# Autodesk Inventor assembly: printer
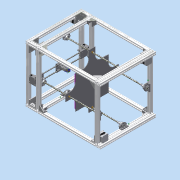
[picture p0: Inventor's stored thumbnail of the model, 180x180]
Saved by Autodesk Inventor 2015 (Build 190159000, 159)
## iProperties
Created: 2016-06-24
Part Number: printer
Document SubType Name: Assembly
Designer: Dustin
Author: Dustin
## Documents named in this file (25)
- E:\Documents\3D Printer\LetzteBot3DPrinter\Inventor Files\IAM Files\printer.iam
- E:\Documents\3D Printer\LetzteBot3DPrinter\Inventor Files\IPT Files\AF350.ipt
- E:\Documents\3D Printer\LetzteBot3DPrinter\Inventor Files\IPT Files\AF380.ipt
- E:\Documents\3D Printer\LetzteBot3DPrinter\Inventor Files\IPT Files\HB1.ipt
- E:\Documents\3D Printer\LetzteBot3DPrinter\Inventor Files\IPT Files\NEMA17.ipt
- E:\Documents\3D Printer\LetzteBot3DPrinter\Inventor Files\IPT Files\LS2.ipt
- E:\Documents\3D Printer\LetzteBot3DPrinter\Inventor Files\IPT Files\LSM1.ipt
- E:\Documents\3D Printer\LetzteBot3DPrinter\Inventor Files\IPT Files\BP1.ipt
- E:\Documents\3D Printer\LetzteBot3DPrinter\Inventor Files\IPT Files\Imported Components\GT2_20teeth_pulley\GT2P.ipt
- E:\Documents\3D Printer\LetzteBot3DPrinter\Inventor Files\IPT Files\SR385.ipt
- E:\Documents\3D Printer\LetzteBot3DPrinter\Inventor Files\IPT Files\MM1.ipt
- E:\Documents\3D Printer\LetzteBot3DPrinter\Inventor Files\IPT Files\AF50.ipt
- E:\Documents\3D Printer\LetzteBot3DPrinter\Inventor Files\IAM Files\extruder.iam
- E:\Documents\3D Printer\LetzteBot3DPrinter\Inventor Files\IPT Files\SM1.ipt
- E:\Documents\3D Printer\LetzteBot3DPrinter\Inventor Files\IPT Files\S320.ipt
- E:\Documents\3D Printer\LetzteBot3DPrinter\Inventor Files\IPT Files\CM1.ipt
- E:\Documents\3D Printer\LetzteBot3DPrinter\Inventor Files\IAM Files\M4BA1.iam
- E:\Documents\3D Printer\LetzteBot3DPrinter\Inventor Files\IAM Files\M4BA2.iam
- E:\Documents\3D Printer\LetzteBot3DPrinter\Inventor Files\IAM Files\KFL08.iam
- E:\Documents\3D Printer\LetzteBot3DPrinter\Inventor Files\IAM Files\VW1.iam
- E:\Documents\3D Printer\LetzteBot3DPrinter\Inventor Files\IPT Files\S516.ipt
- E:\Documents\3D Printer\LetzteBot3DPrinter\Inventor Files\IPT Files\LSN1.ipt
- E:\Documents\3D Printer\LetzteBot3DPrinter\Inventor Files\IPT Files\CB2.ipt
- E:\Documents\3D Printer\LetzteBot3DPrinter\Inventor Files\IPT Files\CM2.ipt
- E:\Documents\3D Printer\LetzteBot3DPrinter\Inventor Files\IPT Files\CB1.ipt
## Components (123 placed, 24 different names)
1. NEMA17:1 — Mate:39, Flush:64, Insert:7, Mate:85, Insert:59
2. NEMA17:2 — Flush:65, Insert:6, Insert:20, Insert:21
3. NEMA17:3 — Mate:87, Mate:88, Insert:32, Insert:60
4. NEMA17:4 — Insert:23, Insert:24, Mate:90, Tangent:34, Insert:31, Mate:98
5. CM1:2 — Flush:91, Mate:101, Angle:14, Tangent:38, Flush:94, Angle:15, Tangent:39, Mate:103
6. MM1:2 — Insert:20, Insert:21, Flush:123
7. MM1:3 — Insert:23, Insert:24, Mate:89
8. MM1:4 — Insert:59, Angle:30
9. MM1:5 — Insert:60, Angle:31, Mate:115
10. CB2:5 — Mate:116, Mate:117, Flush:124
11. CB2:6 — Mate:118, Flush:125, Mate:119
12. CB2:7 — Mate:126, Flush:129, Mate:127
13. CB2:8 — Mate:124, Mate:125, Flush:128
14. CB2:9 — Mate:122, Mate:123, Flush:127
15. CB2:10 — Mate:120, Mate:121, Flush:126
16. CB2:11 — Mate:128, Mate:129, Flush:130
17. CB2:12 — Mate:130, Mate:131, Flush:131
18. CM2:1 — Mate:132, Mate:133, Mate:134
19. CB1:1 — Mate:135, Flush:132, Mate:136
20. CB1:2 — Mate:137, Mate:138, Flush:133
21. CB1:3 — Mate:139, Flush:134, Mate:140
22. CB1:4 — Mate:141, Mate:142, Flush:135
23. CB1:5 — Mate:143, Flush:136, Mate:144
24. CB1:6 — Mate:145, Mate:146, Flush:137
25. CB1:7 — Mate:147, Mate:148, Flush:138
26. CB1:8 — Mate:149, Mate:150, Flush:139
27. CB2:1 — Mate:107, Flush:119, Mate:108
28. CB2:2 — Mate:109, Mate:110, Flush:120
29. CB2:3 — Mate:113, Mate:114, Flush:122
30. CB2:4 — Mate:111, Mate:112, Flush:121
31. AF380:11 — Mate:60, Flush:60, Flush:61
32. AF380:12 — Flush:62, Mate:61, Flush:63
33. AF50:1 — Flush:71, Flush:72, Mate:72, Mate:143, Mate:147
34. AF50:2 — Mate:75, Flush:73, Flush:74, Mate:132, Mate:133, Mate:140, Mate:141, Flush:135, Mate:151, Flush:140
35. AF50:3 — Mate:74, Flush:75, Flush:76, Mate:138, Mate:150, Flush:139
36. AF50:4 — Mate:73, Flush:77, Flush:78, Mate:77, Flush:81, Flush:82, Mate:136, Mate:145
37. AF380:13 — Mate:77, Flush:81, Flush:82, Mate:88, Mate:90, Flush:142
38. AF350:7 — Mate:89, Mate:98, Flush:91, Mate:101, Flush:106, Flush:141, Flush:142
39. AF350:8 — Mate:87, Angle:28, Angle:31, Mate:115, Mate:134
40. AF350:2 — Mate:4, Flush:8, Flush:9, Mate:6, Mate:39, Flush:53, Flush:64, Mate:66, Mate:113, Flush:122, Angle:30
41. AF350:3 — Mate:5, Flush:10, Flush:11, Flush:12, Flush:13, Mate:48, Flush:51, Flush:65, Mate:67, Mate:109, Flush:120
42. AF380:3 — Mate:4, Flush:8, Flush:9, Mate:5, Flush:10, Flush:11, Mate:11, Mate:12, Flush:24, Flush:25, Flush:26, Flush:27, Mate:60, Flush:60, Flush:61, Mate:85, Flush:113, Mate:104, Mate:108
43. AF380:4 — Mate:6, Flush:12, Flush:13, Mate:10, Mate:13, Flush:21, Flush:22, Flush:23, Flush:28, Flush:29, Mate:54, Flush:54, Flush:62, Mate:61, Flush:63, Mate:68, Mate:111, Flush:121, Flush:123
44. AF380:5 — Mate:13, Flush:21, Flush:28, Flush:29, Mate:116, Mate:127
45. AF380:6 — Mate:12, Flush:26, Flush:27, Mate:14, Flush:30, Flush:31, Mate:107, Flush:119, Mate:110, Mate:119, Mate:120
46. AF380:7 — Mate:11, Flush:24, Flush:25, Mate:122, Flush:127, Mate:125
47. AF380:8 — Mate:10, Flush:22, Flush:23, Mate:112, Mate:114, Mate:129, Mate:130, Flush:131
48. AF350:5 — Mate:40, Flush:47, Flush:48, Flush:73, Flush:105, Mate:117, Flush:124, Mate:118, Flush:125, Mate:142, Flush:136, Mate:144
49. AF350:6 — Mate:44, Flush:50, Flush:77, Mate:83, Flush:104, Mate:124, Flush:128, Mate:128, Flush:130, Mate:135, Flush:132, Mate:137, Flush:133
50. AF380:9 — Mate:14, Flush:30, Flush:31, Mate:42, Flush:49, Mate:74, Mate:75, Flush:74, Flush:75, Flush:76, Angle:29, Mate:121, Flush:126, Mate:123, Mate:139, Flush:134, Mate:149
51. AF380:10 — Mate:46, Flush:71, Flush:72, Mate:72, Mate:73, Flush:78, Mate:126, Flush:129, Mate:131, Mate:146, Flush:137, Mate:148, Flush:138
52. AF380:14 — Mate:151, Flush:140, Flush:141
53. LSN1:1 — Insert:50, Tangent:73
54. LSN1:2 — Insert:51, Tangent:74
55. LSN1:3 — Insert:52, Tangent:72, Tangent:75
56. LSN1:4 — Mate:106, Insert:58
57. GT2P:1 — Insert:33
58. GT2P:2 — Insert:5
59. GT2P:3 — Insert:3
60. GT2P:4 — Insert:4
61. GT2P:5 — Insert:6
62. GT2P:6 — Insert:7
63. S320:5 — Insert:54
64. S320:6 — Insert:57
65. S320:7 — Insert:56
66. S320:8 — Insert:55
67. KFL08:1 [sub-assembly] — Flush:109, Tangent:53, Tangent:61
68. KFL08:2 [sub-assembly] — Flush:110, Tangent:55, Tangent:63
69. KFL08:3 [sub-assembly] — Flush:111, Tangent:56, Tangent:57
70. KFL08:4 [sub-assembly] — Flush:112, Tangent:58, Tangent:59
71. KFL08:5 [sub-assembly] — Flush:117, Tangent:68, Tangent:69
72. KFL08:6 [sub-assembly] — Flush:118, Tangent:70, Tangent:71
73. KFL08:7 [sub-assembly] — Flush:116, Tangent:66, Tangent:67
74. KFL08:8 [sub-assembly] — Flush:115, Tangent:64, Tangent:65
75. HB1:1 — Mate:58, Tangent:5, Tangent:6, Insert:54, Insert:55, Insert:56, Insert:57
76. LS2:1 — Tangent:1, Flush:58, Insert:3, Tangent:18, Tangent:24, Tangent:56, Tangent:64
77. LS2:2 — Insert:33, Flush:114, Tangent:62, Tangent:63, Tangent:66, Tangent:75
78. LS2:3 — Tangent:3, Flush:56, Insert:5, Tangent:14, Tangent:58, Tangent:60, Tangent:68
79. LS2:4 — Tangent:2, Flush:55, Insert:4, Tangent:16, Tangent:21, Tangent:53, Tangent:70
80. LSM1:1 — Mate:40, Flush:47, Tangent:1, Flush:111, Tangent:57
81. LSM1:2 — Mate:42, Flush:48, Flush:110, Tangent:55
82. LSM1:3 — Mate:44, Flush:49, Tangent:3, Flush:112, Tangent:59
83. LSM1:4 — Mate:46, Flush:50, Tangent:2, Flush:109, Tangent:61
84. LSM1:5 — Mate:48, Flush:51, Flush:58, Tangent:18, Mate:67, Flush:115, Tangent:65
85. LSM1:6 — Flush:113, Mate:104, Flush:114, Tangent:62, Flush:116, Tangent:67
86. LSM1:7 — Mate:54, Flush:54, Flush:55, Tangent:16, Mate:68, Flush:118, Tangent:71
87. LSM1:8 — Flush:53, Flush:56, Tangent:14, Mate:66, Flush:117, Tangent:69
88. BP1:1 — Mate:58, Tangent:5, Tangent:6, Tangent:21, Tangent:24, Tangent:60, Insert:50, Insert:51, Insert:52, Angle:28, Angle:29, Tangent:72, Tangent:73, Tangent:74, Mate:106, Insert:58
89. S320:1 — Tangent:35, Angle:11, Flush:107
90. S320:2 — Tangent:36, Angle:12, Flush:108
91. S320:3 — Angle:21, Tangent:45, Flush:100
92. S320:4 — Angle:22, Tangent:46, Flush:101
93. S516:1 — Insert:40
94. S516:2 — Insert:41
95. S516:3 — Insert:39
96. S516:4 — Insert:38
97. S516:5 — Insert:46
98. S516:6 — Insert:47
99. S516:7 — Insert:49
100. S516:8 — Insert:48
101. VW1:1 [sub-assembly] — Insert:37
102. VW1:4 [sub-assembly] — Insert:35
103. VW1:3 [sub-assembly] — Insert:36
104. VW1:2 [sub-assembly] — Insert:34
105. VW1:5 [sub-assembly] — Insert:42
106. VW1:6 [sub-assembly] — Insert:43
107. VW1:7 [sub-assembly] — Insert:44
108. VW1:8 [sub-assembly] — Insert:45
109. SR385:1 — Flush:68, Mate:83, Tangent:22, Tangent:47, Tangent:51, Angle:26, Angle:27
110. SR385:2 — Flush:68, Tangent:23, Tangent:48, Angle:25, Tangent:52
111. SM1:1 — Angle:13, Tangent:37, Flush:93, Angle:16, Tangent:40, Flush:95, Tangent:51, Angle:25, Flush:104, Tangent:52, Insert:42, Insert:43, Insert:44, Insert:45, Insert:46, Insert:47, Insert:48, Insert:49
112. SM1:2 — Tangent:47, Tangent:48, Tangent:49, Tangent:50, Angle:23, Angle:24, Flush:102, Flush:103, Angle:26, Flush:105, Insert:34, Insert:35, Insert:36, Insert:37, Insert:38, Insert:39, Insert:40, Insert:41
113. extruder:1 [sub-assembly] — Tangent:22, Tangent:23, Tangent:35, Angle:11, Tangent:36, Angle:12, Angle:21, Tangent:45, Angle:22, Tangent:46, Flush:100, Flush:101, Flush:106, Flush:107, Angle:27, Flush:108
114. M4BA1:1 [sub-assembly] — Angle:13, Tangent:37, Flush:93
115. M4BA1:2 [sub-assembly] — Angle:14, Tangent:38, Flush:94
116. M4BA2:1 [sub-assembly] — Angle:15, Tangent:39, Mate:103
117. M4BA2:2 [sub-assembly] — Angle:16, Tangent:40, Flush:95
118. M4BA1:3 [sub-assembly] — Tangent:50, Angle:24, Flush:103
119. M4BA2:3 [sub-assembly] — Tangent:49, Angle:23, Flush:102
120. M4BA1:4 [sub-assembly]
121. M4BA2:4 [sub-assembly]
122. GT2P:7 — Insert:32
123. GT2P:8 — Tangent:34, Insert:31
## Relationships (287: Flush 98, Mate 85, Tangent 49, Insert 38, Angle 17)
- Mate:4: AF350:2 ↔ AF380:3
- Flush:8: AF350:2 ↔ AF380:3
- Flush:9: AF350:2 ↔ AF380:3
- Mate:5: AF350:3 ↔ AF380:3
- Flush:10: AF350:3 ↔ AF380:3
- Flush:11: AF350:3 ↔ AF380:3
- Mate:6: AF350:2 ↔ AF380:4
- Flush:12: AF350:3 ↔ AF380:4
- Flush:13: AF350:3 ↔ AF380:4
- [Mate]: AF350:6 ↔ AF380:9
- [Flush]: AF350:6 ↔ AF380:9
- [Flush]: AF350:6 ↔ AF380:9
- [Mate]: AF350:5 ↔ AF380:9
- [Flush]: AF350:5 ↔ AF380:9
- [Flush]: AF350:5 ↔ AF380:9
- [Mate]: AF350:6 ↔ AF380:10
- [Flush]: AF350:6 ↔ AF380:10
- [Flush]: AF350:6 ↔ AF380:10
- [Flush]: AF350:5 ↔ AF380:10
- Mate:10: AF380:4 ↔ AF380:8
- Mate:11: AF380:3 ↔ AF380:7
- Mate:12: AF380:3 ↔ AF380:6
- Mate:13: AF380:4 ↔ AF380:5
- Flush:21: AF380:4 ↔ AF380:5
- Flush:22: AF380:4 ↔ AF380:8
- Flush:23: AF380:4 ↔ AF380:8
- Flush:24: AF380:3 ↔ AF380:7
- Flush:25: AF380:3 ↔ AF380:7
- Flush:26: AF380:3 ↔ AF380:6
- Flush:27: AF380:3 ↔ AF380:6
- Flush:28: AF380:4 ↔ AF380:5
- Flush:29: AF380:4 ↔ AF380:5
- Mate:14: AF380:6 ↔ AF380:9
- Flush:30: AF380:6 ↔ AF380:9
- Flush:31: AF380:6 ↔ AF380:9
- Mate:39: NEMA17:1 ↔ AF350:2
- Mate:40: AF350:5 ↔ LSM1:1
- Flush:47: AF350:5 ↔ LSM1:1
- Tangent:1: LS2:1 ↔ LSM1:1
- Mate:42: AF380:9 ↔ LSM1:2
- Flush:48: AF350:5 ↔ LSM1:2
- Mate:44: AF350:6 ↔ LSM1:3
- Flush:49: AF380:9 ↔ LSM1:3
- Mate:46: AF380:10 ↔ LSM1:4
- Flush:50: AF350:6 ↔ LSM1:4
- Tangent:2: LS2:4 ↔ LSM1:4
- Tangent:3: LS2:3 ↔ LSM1:3
- Mate:48: AF350:3 ↔ LSM1:5
- Flush:51: AF350:3 ↔ LSM1:5
- Flush:53: AF350:2 ↔ LSM1:8
- Mate:54: AF380:4 ↔ LSM1:7
- Flush:54: AF380:4 ↔ LSM1:7
- Flush:55 (5 mm): LS2:4 ↔ LSM1:7
- Flush:56 (5 mm): LS2:3 ↔ LSM1:8
- Flush:58 (5 mm): LS2:1 ↔ LSM1:5
- Mate:58 (6 mm): HB1:1 ↔ BP1:1
- Tangent:5: HB1:1 ↔ BP1:1
- Tangent:6: HB1:1 ↔ BP1:1
- Insert:3 (-28 mm): GT2P:3 ↔ LS2:1
- Insert:4 (-28 mm): GT2P:4 ↔ LS2:4
- Insert:5 (-28 mm): GT2P:2 ↔ LS2:3
- Mate:60: AF380:11 ↔ AF380:3
- Flush:60: AF380:11 ↔ AF380:3
- Flush:61: AF380:11 ↔ AF380:3
- Flush:62: AF380:12 ↔ AF380:4
- Mate:61: AF380:12 ↔ AF380:4
- Flush:63: AF380:12 ↔ AF380:4
- Flush:64: NEMA17:1 ↔ AF350:2
- Flush:65: NEMA17:2 ↔ AF350:3
- Insert:6 (-14 mm): NEMA17:2 ↔ GT2P:5
- Insert:7 (-14 mm): NEMA17:1 ↔ GT2P:6
- Flush:68: SR385:1 ↔ SR385:2
- Tangent:14: LS2:3 ↔ LSM1:8
- Tangent:16 (-1 mm): LS2:4 ↔ LSM1:7
- Tangent:18: LS2:1 ↔ LSM1:5
- Mate:66: AF350:2 ↔ LSM1:8
- Mate:67: AF350:3 ↔ LSM1:5
- Mate:68: AF380:4 ↔ LSM1:7
- Flush:71: AF50:1 ↔ AF380:10
- Flush:72: AF50:1 ↔ AF380:10
- Mate:72: AF50:1 ↔ AF380:10
- Mate:73: AF50:4 ↔ AF380:10
- Mate:74: AF50:3 ↔ AF380:9
- Mate:75: AF50:2 ↔ AF380:9
- Flush:73: AF50:2 ↔ AF350:5
- Flush:74: AF50:2 ↔ AF380:9
- Flush:75: AF50:3 ↔ AF380:9
- Flush:76: AF50:3 ↔ AF380:9
- Flush:77: AF50:4 ↔ AF350:6
- Flush:78: AF50:4 ↔ AF380:10
- Mate:77: AF50:4 ↔ AF380:13
- Flush:81: AF50:4 ↔ AF380:13
- Flush:82: AF50:4 ↔ AF380:13
- Insert:20: NEMA17:2 ↔ MM1:2
- Insert:21: NEMA17:2 ↔ MM1:2
- Tangent:21: LS2:4 ↔ BP1:1
- Insert:23: NEMA17:4 ↔ MM1:3
- Insert:24: NEMA17:4 ↔ MM1:3
- Mate:83: AF350:6 ↔ SR385:1
- Tangent:22: SR385:1 ↔ extruder:1
- Tangent:23: SR385:2 ↔ extruder:1
- Mate:85: NEMA17:1 ↔ AF380:3
- Tangent:24: LS2:1 ↔ BP1:1
- Mate:87: NEMA17:3 ↔ AF350:8
- Mate:88: NEMA17:3 ↔ AF380:13
- Mate:89: MM1:3 ↔ AF350:7
- Mate:90: NEMA17:4 ↔ AF380:13
- Tangent:34: NEMA17:4 ↔ GT2P:8
- Insert:31 (5 mm): NEMA17:4 ↔ GT2P:8
- Mate:98: NEMA17:4 ↔ AF350:7
- Tangent:35: S320:1 ↔ extruder:1
- Angle:11 (180 deg): S320:1 ↔ extruder:1
- Flush:91: CM1:2 ↔ AF350:7
- Mate:101: CM1:2 ↔ AF350:7
- Insert:32: NEMA17:3 ↔ GT2P:7
- Tangent:36: S320:2 ↔ extruder:1
- Angle:12 (180 deg): S320:2 ↔ extruder:1
- Angle:13 (180 deg): SM1:1 ↔ M4BA1:1
- Tangent:37: SM1:1 ↔ M4BA1:1
- Flush:93 (-5 mm): SM1:1 ↔ M4BA1:1
- Angle:14 (0 deg): CM1:2 ↔ M4BA1:2
- Tangent:38: CM1:2 ↔ M4BA1:2
- Flush:94 (-6 mm): CM1:2 ↔ M4BA1:2
- Angle:15 (0 deg): CM1:2 ↔ M4BA2:1
- Tangent:39: CM1:2 ↔ M4BA2:1
- Mate:103 (15 mm): CM1:2 ↔ M4BA2:1
- Angle:16 (180 deg): SM1:1 ↔ M4BA2:2
- Tangent:40: SM1:1 ↔ M4BA2:2
- Flush:95: SM1:1 ↔ M4BA2:2
- Angle:21 (180 deg): S320:3 ↔ extruder:1
- Tangent:45: S320:3 ↔ extruder:1
- Angle:22 (180 deg): S320:4 ↔ extruder:1
- Tangent:46: S320:4 ↔ extruder:1
- Flush:100 (-6 mm): S320:3 ↔ extruder:1
- Flush:101 (-2 mm): S320:4 ↔ extruder:1
- Tangent:47: SR385:1 ↔ SM1:2
- Tangent:48: SR385:2 ↔ SM1:2
- Tangent:49: SM1:2 ↔ M4BA2:3
- Tangent:50: SM1:2 ↔ M4BA1:3
- Angle:23 (180 deg): SM1:2 ↔ M4BA2:3
- Angle:24 (180 deg): SM1:2 ↔ M4BA1:3
- Flush:102 (1 mm): SM1:2 ↔ M4BA2:3
- Flush:103 (-5 mm): SM1:2 ↔ M4BA1:3
- Tangent:51: SR385:1 ↔ SM1:1
- Angle:25 (0 deg): SR385:2 ↔ SM1:1
- Flush:104: AF350:6 ↔ SM1:1
- Tangent:52: SR385:2 ↔ SM1:1
- Angle:26 (0 deg): SR385:1 ↔ SM1:2
- Flush:105: AF350:5 ↔ SM1:2
- Flush:106 (47 mm): AF350:7 ↔ extruder:1
- Flush:107: S320:1 ↔ extruder:1
- Angle:27 (0 deg): SR385:1 ↔ extruder:1
- Flush:108 (-5 mm): S320:2 ↔ extruder:1
- Flush:109: KFL08:1 ↔ LSM1:4
- Tangent:53: KFL08:1 ↔ LS2:4
- Flush:110: KFL08:2 ↔ LSM1:2
- Tangent:55: KFL08:2 ↔ LSM1:2
- Flush:111: KFL08:3 ↔ LSM1:1
- Tangent:56: KFL08:3 ↔ LS2:1
- Tangent:57: KFL08:3 ↔ LSM1:1
- Flush:112: KFL08:4 ↔ LSM1:3
- Tangent:58: KFL08:4 ↔ LS2:3
- Tangent:59: KFL08:4 ↔ LSM1:3
- Tangent:60 (-1 mm): LS2:3 ↔ BP1:1
- Tangent:61: KFL08:1 ↔ LSM1:4
- Flush:113: AF380:3 ↔ LSM1:6
- Mate:104: AF380:3 ↔ LSM1:6
- Insert:33 (-23 mm): GT2P:1 ↔ LS2:2
- Flush:114 (-5 mm): LS2:2 ↔ LSM1:6
- Tangent:62: LS2:2 ↔ LSM1:6
- Tangent:63: KFL08:2 ↔ LS2:2
- Flush:115: KFL08:8 ↔ LSM1:5
- Tangent:64: KFL08:8 ↔ LS2:1
- Tangent:65: KFL08:8 ↔ LSM1:5
- Flush:116: KFL08:7 ↔ LSM1:6
- Tangent:66: KFL08:7 ↔ LS2:2
- Tangent:67: KFL08:7 ↔ LSM1:6
- Flush:117: KFL08:5 ↔ LSM1:8
- Tangent:68: KFL08:5 ↔ LS2:3
- Tangent:69: KFL08:5 ↔ LSM1:8
- Flush:118: KFL08:6 ↔ LSM1:7
- Tangent:70: KFL08:6 ↔ LS2:4
- Tangent:71: KFL08:6 ↔ LSM1:7
- Insert:34 (0.4 mm): VW1:2 ↔ SM1:2
- Insert:35 (0.4 mm): VW1:4 ↔ SM1:2
- Insert:36 (0.4 mm): VW1:3 ↔ SM1:2
- Insert:37 (0.4 mm): VW1:1 ↔ SM1:2
- Insert:38: S516:4 ↔ SM1:2
- Insert:39: S516:3 ↔ SM1:2
- Insert:40: S516:1 ↔ SM1:2
- Insert:41: S516:2 ↔ SM1:2
- Insert:42: VW1:5 ↔ SM1:1
- Insert:43: VW1:6 ↔ SM1:1
- Insert:44: VW1:7 ↔ SM1:1
- Insert:45: VW1:8 ↔ SM1:1
- Insert:46: S516:5 ↔ SM1:1
- Insert:47: S516:6 ↔ SM1:1
- Insert:48: S516:8 ↔ SM1:1
- Insert:49: S516:7 ↔ SM1:1
- Insert:50: LSN1:1 ↔ BP1:1
- Insert:51: LSN1:2 ↔ BP1:1
- Insert:52: LSN1:3 ↔ BP1:1
- Angle:28 (0 deg): AF350:8 ↔ BP1:1
- Angle:29 (0 deg): AF380:9 ↔ BP1:1
- Insert:54: S320:5 ↔ HB1:1
- Insert:55: S320:8 ↔ HB1:1
- Insert:56: S320:7 ↔ HB1:1
- Insert:57: S320:6 ↔ HB1:1
- Tangent:72: LSN1:3 ↔ BP1:1
- Tangent:73: LSN1:1 ↔ BP1:1
- Tangent:74: LSN1:2 ↔ BP1:1
- Mate:106: LSN1:4 ↔ BP1:1
- Insert:58: LSN1:4 ↔ BP1:1
- Mate:107: CB2:1 ↔ AF380:6
- Flush:119: CB2:1 ↔ AF380:6
- Mate:108: CB2:1 ↔ AF380:3
- Mate:109: CB2:2 ↔ AF350:3
- Mate:110: CB2:2 ↔ AF380:6
- Flush:120: CB2:2 ↔ AF350:3
- Mate:111: CB2:4 ↔ AF380:4
- Mate:112: CB2:4 ↔ AF380:8
- Flush:121: CB2:4 ↔ AF380:4
- Mate:113: CB2:3 ↔ AF350:2
- Mate:114: CB2:3 ↔ AF380:8
- Flush:122: CB2:3 ↔ AF350:2
- Flush:123: MM1:2 ↔ AF380:4
- Insert:59: NEMA17:1 ↔ MM1:4
- Angle:30 (0 deg): MM1:4 ↔ AF350:2
- Insert:60: NEMA17:3 ↔ MM1:5
- Angle:31 (0 deg): MM1:5 ↔ AF350:8
- Mate:115: MM1:5 ↔ AF350:8
- Mate:116: CB2:5 ↔ AF380:5
- Mate:117: CB2:5 ↔ AF350:5
- Flush:124: CB2:5 ↔ AF350:5
- Mate:118: CB2:6 ↔ AF350:5
- Flush:125: CB2:6 ↔ AF350:5
- Mate:119: CB2:6 ↔ AF380:6
- Mate:120: CB2:10 ↔ AF380:6
- Mate:121: CB2:10 ↔ AF380:9
- Flush:126: CB2:10 ↔ AF380:9
- Mate:122: CB2:9 ↔ AF380:7
- Mate:123: CB2:9 ↔ AF380:9
- Flush:127: CB2:9 ↔ AF380:7
- Mate:124: CB2:8 ↔ AF350:6
- Mate:125: CB2:8 ↔ AF380:7
- Flush:128: CB2:8 ↔ AF350:6
- Mate:126: CB2:7 ↔ AF380:10
- Flush:129: CB2:7 ↔ AF380:10
- Mate:127: CB2:7 ↔ AF380:5
- Mate:128: CB2:11 ↔ AF350:6
- Mate:129: CB2:11 ↔ AF380:8
- Flush:130: CB2:11 ↔ AF350:6
- Mate:130: CB2:12 ↔ AF380:8
- Mate:131: CB2:12 ↔ AF380:10
- Flush:131: CB2:12 ↔ AF380:8
- Mate:132: CM2:1 ↔ AF50:2
- Mate:133: CM2:1 ↔ AF50:2
- Mate:134: CM2:1 ↔ AF350:8
- Mate:135: CB1:1 ↔ AF350:6
- Flush:132: CB1:1 ↔ AF350:6
- Mate:136: CB1:1 ↔ AF50:4
- Mate:137: CB1:2 ↔ AF350:6
- Mate:138: CB1:2 ↔ AF50:3
- Flush:133: CB1:2 ↔ AF350:6
- Mate:139: CB1:3 ↔ AF380:9
- Flush:134: CB1:3 ↔ AF380:9
- Mate:140: CB1:3 ↔ AF50:2
- Mate:141: CB1:4 ↔ AF50:2
- Mate:142: CB1:4 ↔ AF350:5
- Flush:135: CB1:4 ↔ AF50:2
- Mate:143: CB1:5 ↔ AF50:1
- Flush:136: CB1:5 ↔ AF350:5
- Mate:144: CB1:5 ↔ AF350:5
- Mate:145: CB1:6 ↔ AF50:4
- Mate:146: CB1:6 ↔ AF380:10
- Flush:137: CB1:6 ↔ AF380:10
- Mate:147: CB1:7 ↔ AF50:1
- Mate:148: CB1:7 ↔ AF380:10
- Flush:138: CB1:7 ↔ AF380:10
- Mate:149: CB1:8 ↔ AF380:9
- Mate:150: CB1:8 ↔ AF50:3
- Flush:139: CB1:8 ↔ AF50:3
- Tangent:75: LSN1:3 ↔ LS2:2
- Mate:151: AF50:2 ↔ AF380:14
- Flush:140: AF50:2 ↔ AF380:14
- Flush:141: AF350:7 ↔ AF380:14
- Flush:142: AF380:13 ↔ AF350:7
## Named parameters: d25_d15 = 0 mm, d26_d6 = 0 mm, d27_d7 = 0 mm, d28_d8 = 0 mm, d29_d9 = 0 mm, d30_d10 = 0 mm, d31_d11 = 0 mm, d32_d12 = 0 mm, d33_d13 = 0 mm, d34_d14 = 0 mm
